# Autodesk Inventor assembly: Complete Divider
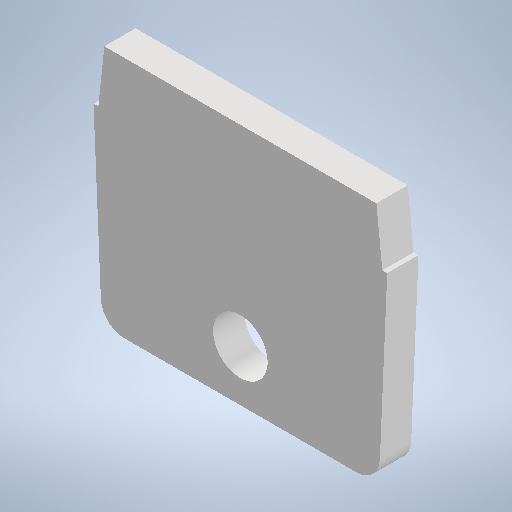
[picture p0: Inventor's stored thumbnail of the model, 512x512]
Saved by Autodesk Inventor 2025 (Build 290162010, 162A)
## iProperties
Created: 2024-10-17
Part Number: Complete Divider
Document SubType Name: Assembly
Designer: vncnt
Author: vncnt
## Documents named in this file (3)
- C:\Users\vncnt\City Tech Dropbox\Vincent Ching\Neuroscience\Mouse city\CAD\ASRC NeuroScience Mouse Experiment\Complete Divider.iam
- C:\Users\vncnt\City Tech Dropbox\Vincent Ching\Neuroscience\Mouse city\CAD\ASRC NeuroScience Mouse Experiment\Divider.ipt
- C:\Users\vncnt\City Tech Dropbox\Vincent Ching\Neuroscience\Mouse city\CAD\ASRC NeuroScience Mouse Experiment\Lid_Divider.ipt
## Components (2 placed, 2 different names)
1. Divider:1 — Mate:1, Flush:1
2. Lid_Divider:1 — Mate:1, Flush:1
## Relationships (2: Mate 1, Flush 1)
- Mate:1: Divider:1 ↔ Lid_Divider:1
- Flush:1: Divider:1 ↔ Lid_Divider:1
